# Autodesk Inventor assembly: mx28_withHorn
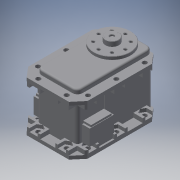
[picture p0: Inventor's stored thumbnail of the model, 180x180]
Saved by Autodesk Inventor 2016 (Build 200138000, 138)
## iProperties
Created: 2014-04-23
Part Number: mx28_withHorn
Document SubType Name: Assembly
Designer: BitBots
Author: BitBots
## Documents named in this file (3)
- C:\Hambot\motors\MX28\mx28_with_horn.iam
- C:\Hambot\motors\MX28\mx28_body.ipt
- C:\Hambot\motors\MX28\HN07-N101.ipt
## Components (2 placed, 2 different names)
1. mx28_body:1 — Rotational:2
2. HN07-N101:1 — Rotational:2
## Relationships (1: RevoluteJoint 1)
- Rotational:2 [RevoluteJoint]: mx28_body:1 ↔ HN07-N101:1
